# Autodesk Inventor assembly: Group
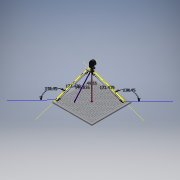
[picture p0: Inventor's stored thumbnail of the model, 180x180]
Saved by Autodesk Inventor 2018.2 (Build 222227000, 227)
## iProperties
Created: 2018-04-10
Part Number: Group
Material: Generisch
Document SubType Name: Assembly
Designer: Nick Koch
Author: Nick Koch
## Documents named in this file (6)
- C:\Users\Nick Koch\Desktop\Lehre\FHNW\Raytracing Modell\v2\Group.iam
- C:\Users\Nick Koch\Desktop\Lehre\FHNW\Raytracing Modell\v2\MiddleStick.ipt
- C:\Users\Nick Koch\Desktop\Lehre\FHNW\Raytracing Modell\v2\Screen.ipt
- C:\Users\Nick Koch\Desktop\Lehre\FHNW\Raytracing Modell\v2\Camera.ipt
- C:\Users\Nick Koch\Desktop\Lehre\FHNW\Raytracing Modell\v2\blueStick.ipt
- C:\Users\Nick Koch\Desktop\Lehre\FHNW\Raytracing Modell\v2\FOVStick.ipt
## Components (6 placed, 5 different names)
1. MiddleStick:1 — Passend:1, Passend:2, Passend:3, Passend:4, Passend:5, Passend:6, Passend:16
2. Screen:1 — Passend:1, Passend:2, Passend:3, Passend:16
3. Camera:1 — Passend:4, Passend:5, Passend:6, Passend:13, Passend:14, Passend:15, Passend:19, Passend:20, Passend:21
4. blueStick:3 — Passend:13, Passend:14, Passend:15
5. FOVStick:2 — Passend:21
6. FOVStick:3
## Relationships (13: Mate 13)
- Passend:1 [Mate]: MiddleStick:1 ↔ Screen:1
- Passend:2 [Mate]: MiddleStick:1 ↔ Screen:1
- Passend:3 [Mate]: MiddleStick:1 ↔ Screen:1
- Passend:4 [Mate]: MiddleStick:1 ↔ Camera:1
- Passend:5 [Mate]: MiddleStick:1 ↔ Camera:1
- Passend:6 [Mate]: MiddleStick:1 ↔ Camera:1
- Passend:13 [Mate]: Camera:1 ↔ blueStick:3
- Passend:14 [Mate]: Camera:1 ↔ blueStick:3
- Passend:15 [Mate]: Camera:1 ↔ blueStick:3
- Passend:16 [Mate]: MiddleStick:1 ↔ Screen:1
- Passend:19 [Mate]: Camera:1
- Passend:20 [Mate]: Camera:1
- Passend:21 [Mate]: Camera:1 ↔ FOVStick:2
